# Autodesk Inventor assembly: k2
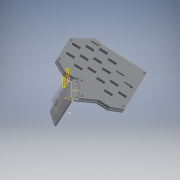
[picture p0: Inventor's stored thumbnail of the model, 180x180]
Saved by Autodesk Inventor 2017 (Build 210142000, 142)
## iProperties
Created: 2017-02-07
Part Number: k2
Document SubType Name: Assembly
Designer: herman
Author: herman
## Documents named in this file (12)
- C:\Users\herman\Documents\keyboard2\k2.iam
- C:\Users\herman\Documents\keyboard2\k2_l1.ipt
- C:\Users\herman\Documents\keyboard2\k2_l4.ipt
- C:\Users\herman\Documents\keyboard2\k2_l3.ipt
- C:\Users\herman\Documents\keyboard2\k2_l2.ipt
- C:\Users\herman\Documents\keyboard2\k2_t2_l4.ipt
- C:\Users\herman\Documents\keyboard2\k2_t2_l3.ipt
- C:\Users\herman\Documents\keyboard2\k2_t2_l1.ipt
- C:\Users\herman\Documents\keyboard2\k2_hinge1_bot.ipt
- C:\Users\herman\Documents\keyboard2\k2_hinge1_top.ipt
- C:\Users\herman\Documents\keyboard2\k2_feet.ipt
- C:\Users\herman\Documents\keyboard2\k2_t_leg.ipt
## Components (13 placed, 11 different names)
1. k2_l4:1 — Mate:1, Mate:2, Mate:16
2. k2_l3:1 — Mate:1, Mate:2, Mate:3, Mate:4, Mate:15
3. k2_l2:1 — Mate:3, Mate:4, Mate:5, Mate:6
4. k2_l1:1 — Mate:5, Mate:6, Mate:33, Mate:34
5. k2_t2_l3:1 — Mate:20, Mate:21, Mate:22, Mate:25, Mate:26, Mate:27, Mate:28, Mate:30, Mate:32
6. k2_t2_l1:1 — Mate:21, Mate:22, Mate:23, Mate:24
7. k2_hinge1_bot:1 — Rotational:1, Mate:20, Mate:29, Mate:32
8. k2_hinge1_top:1 — Mate:15, Mate:16, Rotational:1
9. k2_t2_l1:2 — Mate:23, Mate:24
10. k2_feet:1 — Mate:25, Mate:26, Mate:30, Mate:31
11. k2_t2_l4:1 — Mate:27, Mate:28, Mate:29, Mate:31
12. k2_t_leg:1 — Mate:33, Mate:34, Mate:35, Mate:36
13. k2_t_leg:2 — Mate:35, Mate:36
## Relationships (26: Mate 25, RevoluteJoint 1)
- Mate:1: k2_l4:1 ↔ k2_l3:1
- Mate:2: k2_l4:1 ↔ k2_l3:1
- Mate:3: k2_l3:1 ↔ k2_l2:1
- Mate:4: k2_l3:1 ↔ k2_l2:1
- Mate:5: k2_l2:1 ↔ k2_l1:1
- Mate:6: k2_l2:1 ↔ k2_l1:1
- Mate:15: k2_l3:1 ↔ k2_hinge1_top:1
- Mate:16: k2_l4:1 ↔ k2_hinge1_top:1
- Rotational:1 [RevoluteJoint]: k2_hinge1_bot:1 ↔ k2_hinge1_top:1
- Mate:20: k2_t2_l3:1 ↔ k2_hinge1_bot:1
- Mate:21: k2_t2_l3:1 ↔ k2_t2_l1:1
- Mate:22: k2_t2_l3:1 ↔ k2_t2_l1:1
- Mate:23: k2_t2_l1:1 ↔ k2_t2_l1:2
- Mate:24: k2_t2_l1:1 ↔ k2_t2_l1:2
- Mate:25: k2_t2_l3:1 ↔ k2_feet:1
- Mate:26: k2_t2_l3:1 ↔ k2_feet:1
- Mate:27: k2_t2_l3:1 ↔ k2_t2_l4:1
- Mate:28: k2_t2_l3:1 ↔ k2_t2_l4:1
- Mate:29: k2_hinge1_bot:1 ↔ k2_t2_l4:1
- Mate:30: k2_t2_l3:1 ↔ k2_feet:1
- Mate:31: k2_feet:1 ↔ k2_t2_l4:1
- Mate:32: k2_t2_l3:1 ↔ k2_hinge1_bot:1
- Mate:33: k2_l1:1 ↔ k2_t_leg:1
- Mate:34: k2_l1:1 ↔ k2_t_leg:1
- Mate:35: k2_t_leg:1 ↔ k2_t_leg:2
- Mate:36: k2_t_leg:1 ↔ k2_t_leg:2
